# Autodesk Inventor assembly: Montagem Atualizada
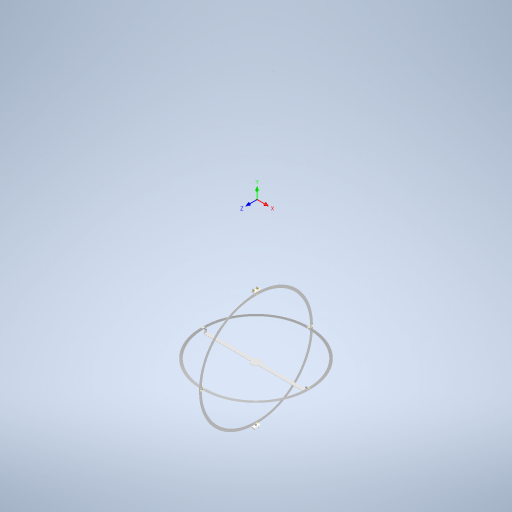
[picture p0: Inventor's stored thumbnail of the model, 512x512]
Saved by Autodesk Inventor 2024 (Build 280153000, 153)
## iProperties
Created: 2024-05-09
Part Number: Montagem Atualizada
Document SubType Name: Assembly
Designer: mathe
Author: mathe
## Documents named in this file (18)
- C:\Users\mathe\OneDrive\Área de Trabalho\Plataforma de Testes\Montagem Atualizada.iam
- C:\Users\mathe\OneDrive\Área de Trabalho\Plataforma de Testes\Suporte Central Atualizado.ipt
- C:\Users\mathe\OneDrive\Documentos\Inventor\Content Center Files\R2024\pt-BR\BS 290 SKF(19)\BS 290 SKF - SKF 108.ipt
- C:\Users\mathe\OneDrive\Área de Trabalho\Plataforma de Testes\Abraçadeira.ipt
- C:\Users\mathe\OneDrive\Área de Trabalho\Plataforma de Testes\Arco menor.ipt
- C:\Users\mathe\OneDrive\Documentos\Inventor\Content Center Files\R2024\pt-BR\BS EN 22 338  C - W\ISO 2338 - 8 h11 x 60 - CBS EN.ipt
- C:\Users\mathe\OneDrive\Documentos\Inventor\Content Center Files\R2024\pt-BR\BS 4183(5)\BS 4183 - M5 x 20(2) I.ipt
- C:\Users\mathe\OneDrive\Documentos\Inventor\Content Center Files\R2024\pt-BR\ANSI B18.2.4.2M\ANSI B18.2.4.2M - M5x0,8 - 8.ipt
- C:\Users\mathe\OneDrive\Área de Trabalho\Plataforma de Testes\Abraçadeira_CPY1.ipt
- C:\Users\mathe\OneDrive\Área de Trabalho\Plataforma de Testes\Abraçadeira_CPY1_CPY.ipt
- C:\Users\mathe\OneDrive\Área de Trabalho\Plataforma de Testes\Abraçadeira_CPY1_CPY_CPY.ipt
- C:\Users\mathe\OneDrive\Área de Trabalho\Plataforma de Testes\Arco médio.ipt
- C:\Users\mathe\OneDrive\Área de Trabalho\Plataforma de Testes\Abraçadeira_CPY1_CPY_CPY1.ipt
- C:\Users\mathe\OneDrive\Área de Trabalho\Plataforma de Testes\Abraçadeira_CPY1_CPY_CPY1_CPY.ipt
- C:\Users\mathe\OneDrive\Área de Trabalho\Plataforma de Testes\Suporte para estrutura_CPY.ipt
- C:\Users\mathe\OneDrive\Área de Trabalho\Plataforma de Testes\Pecinha do perfil.ipt
- C:\Users\mathe\OneDrive\Área de Trabalho\Plataforma de Testes\Suporte para estrutura_CPY_CPY1.ipt
- C:\Users\mathe\OneDrive\Área de Trabalho\Plataforma de Testes\Pecinha do perfil_CPY.ipt
## Components (73 placed, 17 different names)
1. Suporte Central Atualizado:1 — Coincidente:1, Coincidente:4, Coincidente:5, Coincidente:9, Coincidente:66, Coincidente:71, Ângulo:1
2. BS 290 SKF- com furo cilíndrico SKF 108:1 — Coincidente:1, Coincidente:3, Coincidente:70
3. BS 290 SKF- com furo cilíndrico SKF 108:2 — Coincidente:5, Coincidente:66, Coincidente:67
4. Abraçadeira:1 — Coincidente:7, Coincidente:8, Coincidente:10, Coincidente:11, Coincidente:13, Coincidente:14, Coincidente:15, Coincidente:17, Coincidente:18, Coincidente:19, Coincidente:20, Coincidente:21, Coincidente:65, Coincidente:70
5. BS 290 SKF- com furo cilíndrico SKF 108:3 — Coincidente:3, Coincidente:4
6. Arco menor:1 — Coincidente:7, Coincidente:8, Coincidente:17, Coincidente:47, Coincidente:48
7. BS EN 22338 C - extraído 8 h11 x 60 - C:1 — Coincidente:9, Coincidente:65
8. BS 4183 Parafuso de fenda de máquina de cabeça cilíndrica - Métrica M5 x 20:2 — Coincidente:10, Coincidente:11, Coincidente:12
9. ANSI B18.2.4.2M M5x0,8:1 — Coincidente:12, Coincidente:13
10. Arco menor:2 — Coincidente:33, Coincidente:34, Coincidente:49, Coincidente:50
11. Arco menor:3 — Coincidente:35, Coincidente:36, Coincidente:61, Coincidente:63, Ângulo:2
12. Arco menor:4 — Coincidente:14, Coincidente:15, Coincidente:18, Coincidente:62, Coincidente:64
13. BS 4183 Parafuso de fenda de máquina de cabeça cilíndrica - Métrica M5 x 20:3 — Coincidente:19, Coincidente:20, Coincidente:22
14. ANSI B18.2.4.2M M5x0,8:2 — Coincidente:21, Coincidente:22
15. BS 290 SKF- com furo cilíndrico SKF 108:4 — Coincidente:23, Coincidente:24, Coincidente:68
16. Abraçadeira_CPY1:1 — Coincidente:23, Coincidente:24, Coincidente:25, Coincidente:26, Coincidente:27, Coincidente:29, Coincidente:30, Coincidente:32, Coincidente:34, Coincidente:36, Coincidente:69, Coincidente:71
17. BS 4183 Parafuso de fenda de máquina de cabeça cilíndrica - Métrica M5 x 20:4 — Coincidente:25, Coincidente:26, Coincidente:28, Coincidente:33
18. ANSI B18.2.4.2M M5x0,8:3 — Coincidente:27, Coincidente:28
19. BS 4183 Parafuso de fenda de máquina de cabeça cilíndrica - Métrica M5 x 20:5 — Coincidente:29, Coincidente:30, Coincidente:31, Coincidente:35
20. ANSI B18.2.4.2M M5x0,8:4 — Coincidente:31, Coincidente:32
21. BS 290 SKF- com furo cilíndrico SKF 108:5 — Coincidente:72, Coincidente:76, Coincidente:77, Coincidente:144
22. Abraçadeira_CPY1_CPY:1 — Coincidente:39, Coincidente:40, Coincidente:42, Coincidente:43, Coincidente:44, Coincidente:45, Coincidente:48, Coincidente:50, Coincidente:76, Coincidente:77, Coincidente:146
23. BS 4183 Parafuso de fenda de máquina de cabeça cilíndrica - Métrica M5 x 20:6 — Coincidente:39, Coincidente:40, Coincidente:41, Coincidente:49
24. ANSI B18.2.4.2M M5x0,8:5 — Coincidente:41, Coincidente:42
25. BS 4183 Parafuso de fenda de máquina de cabeça cilíndrica - Métrica M5 x 20:7 — Coincidente:43, Coincidente:44, Coincidente:46, Coincidente:47
26. ANSI B18.2.4.2M M5x0,8:6 — Coincidente:45, Coincidente:46
27. BS 290 SKF- com furo cilíndrico SKF 108:6 — Coincidente:51, Coincidente:52, Coincidente:145
28. Abraçadeira_CPY1_CPY_CPY:1 — Coincidente:51, Coincidente:52, Coincidente:53, Coincidente:54, Coincidente:55, Coincidente:57, Coincidente:58, Coincidente:60, Coincidente:63, Coincidente:64
29. BS 4183 Parafuso de fenda de máquina de cabeça cilíndrica - Métrica M5 x 20:8 — Coincidente:53, Coincidente:54, Coincidente:56, Coincidente:61
30. ANSI B18.2.4.2M M5x0,8:7 — Coincidente:55, Coincidente:56
31. BS 4183 Parafuso de fenda de máquina de cabeça cilíndrica - Métrica M5 x 20:9 — Coincidente:57, Coincidente:58, Coincidente:59, Coincidente:62
32. ANSI B18.2.4.2M M5x0,8:8 — Coincidente:59, Coincidente:60
33. BS EN 22338 C - extraído 8 h11 x 60 - C:2 — Coincidente:67, Coincidente:68, Coincidente:69
34. BS EN 22338 C - extraído 8 h11 x 60 - C:3 — Coincidente:72
35. Arco médio:1 — Coincidente:90, Coincidente:91, Coincidente:141, Ângulo:5
36. Arco médio:2 — Coincidente:119, Coincidente:120, Coincidente:142, Coincidente:143, Ângulo:3, Ângulo:4, Ângulo:11
37. Arco médio:3 — Coincidente:103, Coincidente:105, Coincidente:117, Coincidente:118
38. Arco médio:5 — Coincidente:88, Coincidente:89, Coincidente:102, Coincidente:104
39. BS 290 SKF- com furo cilíndrico SKF 108:7 — Coincidente:78, Coincidente:79, Coincidente:155
40. Abraçadeira_CPY1_CPY:2 — Coincidente:78, Coincidente:79, Coincidente:80, Coincidente:81, Coincidente:83, Coincidente:84, Coincidente:85, Coincidente:86, Coincidente:89, Coincidente:90, Coincidente:156
41. BS 4183 Parafuso de fenda de máquina de cabeça cilíndrica - Métrica M5 x 20:10 — Coincidente:80, Coincidente:81, Coincidente:82, Coincidente:91
42. ANSI B18.2.4.2M M5x0,8:9 — Coincidente:82, Coincidente:83
43. BS 4183 Parafuso de fenda de máquina de cabeça cilíndrica - Métrica M5 x 20:11 — Coincidente:84, Coincidente:85, Coincidente:87, Coincidente:88
44. ANSI B18.2.4.2M M5x0,8:10 — Coincidente:86, Coincidente:87
45. BS 290 SKF- com furo cilíndrico SKF 108:8 — Coincidente:92, Coincidente:93, Coincidente:145, Coincidente:148
46. Abraçadeira_CPY1_CPY_CPY1:1 — Coincidente:92, Coincidente:93, Coincidente:94, Coincidente:95, Coincidente:96, Coincidente:98, Coincidente:99, Coincidente:101, Coincidente:104, Coincidente:105, Coincidente:147
47. BS 4183 Parafuso de fenda de máquina de cabeça cilíndrica - Métrica M5 x 20:12 — Coincidente:94, Coincidente:95, Coincidente:97, Coincidente:102
48. ANSI B18.2.4.2M M5x0,8:11 — Coincidente:96, Coincidente:97
49. BS 4183 Parafuso de fenda de máquina de cabeça cilíndrica - Métrica M5 x 20:13 — Coincidente:98, Coincidente:99, Coincidente:100, Coincidente:103
50. ANSI B18.2.4.2M M5x0,8:12 — Coincidente:100, Coincidente:101
51. BS 290 SKF- com furo cilíndrico SKF 108:9 — Coincidente:121, Coincidente:122, Coincidente:172
52. Abraçadeira_CPY1_CPY_CPY1_CPY:1 — Coincidente:108, Coincidente:109, Coincidente:111, Coincidente:112, Coincidente:113, Coincidente:114, Coincidente:118, Coincidente:120, Coincidente:121, Coincidente:122, Coincidente:195
53. BS 4183 Parafuso de fenda de máquina de cabeça cilíndrica - Métrica M5 x 20:14 — Coincidente:108, Coincidente:109, Coincidente:110, Coincidente:119
54. ANSI B18.2.4.2M M5x0,8:13 — Coincidente:110, Coincidente:111
55. BS 4183 Parafuso de fenda de máquina de cabeça cilíndrica - Métrica M5 x 20:15 — Coincidente:112, Coincidente:113, Coincidente:115, Coincidente:117
56. ANSI B18.2.4.2M M5x0,8:14 — Coincidente:114, Coincidente:115
57. BS 290 SKF- com furo cilíndrico SKF 108:10 — Coincidente:123, Coincidente:124, Coincidente:144
58. Abraçadeira_CPY1_CPY_CPY1:2 — Coincidente:123, Coincidente:124, Coincidente:125, Coincidente:126, Coincidente:127, Coincidente:129, Coincidente:130, Coincidente:132, Coincidente:143, Coincidente:146
59. BS 4183 Parafuso de fenda de máquina de cabeça cilíndrica - Métrica M5 x 20:16 — Coincidente:125, Coincidente:126, Coincidente:128, Coincidente:142
60. ANSI B18.2.4.2M M5x0,8:15 — Coincidente:127, Coincidente:128
61. BS 4183 Parafuso de fenda de máquina de cabeça cilíndrica - Métrica M5 x 20:17 — Coincidente:129, Coincidente:130, Coincidente:131, Coincidente:141
62. ANSI B18.2.4.2M M5x0,8:16 — Coincidente:131, Coincidente:132
63. BS EN 22338 C - extraído 8 h11 x 60 - C:4 — Coincidente:147, Coincidente:148
64. BS 290 SKF- com furo cilíndrico SKF 108:12 — Coincidente:174, Coincidente:175, Coincidente:176
65. BS EN 22338 C - extraído 8 h11 x 60 - C:7 — Coincidente:155, Coincidente:156, Coincidente:174, Coincidente:175, Coincidente:177
66. Suporte para estrutura_CPY:2 — Coincidente:176, Coincidente:177, Ângulo:5, Coincidente:178, Coincidente:179, Ângulo:7, Coincidente:180, Coincidente:181, Ângulo:8
67. BS EN 22338 C - extraído 8 h11 x 60 - C:8 — Coincidente:172, Coincidente:187, Coincidente:190
68. Pecinha do perfil:1 — Coincidente:178, Coincidente:179, Ângulo:7
69. Pecinha do perfil:2 — Coincidente:180, Coincidente:181, Ângulo:8
70. BS 290 SKF- com furo cilíndrico SKF 108:13 — Coincidente:189, Coincidente:190, Coincidente:194
71. Suporte para estrutura_CPY_CPY1:1 — Ângulo:9, Coincidente:183, Coincidente:184, Ângulo:10, Coincidente:185, Coincidente:186, Coincidente:187, Coincidente:189, Ângulo:11, Coincidente:194, Coincidente:195
72. Pecinha do perfil_CPY:1 — Ângulo:9, Coincidente:183, Coincidente:184
73. Pecinha do perfil_CPY:2 — Ângulo:10, Coincidente:185, Coincidente:186
## Relationships (161: Mate 151, Angle 10)
- Coincidente:1 [Mate]: Suporte Central Atualizado:1 ↔ BS 290 SKF- com furo cilíndrico SKF 108:1
- Coincidente:3 [Mate]: BS 290 SKF- com furo cilíndrico SKF 108:1 ↔ BS 290 SKF- com furo cilíndrico SKF 108:3
- Coincidente:4 [Mate]: Suporte Central Atualizado:1 ↔ BS 290 SKF- com furo cilíndrico SKF 108:3
- Coincidente:5 [Mate]: Suporte Central Atualizado:1 ↔ BS 290 SKF- com furo cilíndrico SKF 108:2
- Coincidente:7 [Mate]: Abraçadeira:1 ↔ Arco menor:1
- Coincidente:8 [Mate]: Abraçadeira:1 ↔ Arco menor:1
- Coincidente:9 [Mate]: Suporte Central Atualizado:1 ↔ BS EN 22338 C - extraído 8 h11 x 60 - C:1
- Coincidente:10 [Mate]: Abraçadeira:1 ↔ BS 4183 Parafuso de fenda de máquina de cabeça cilíndrica - Métrica M5 x 20:2
- Coincidente:11 [Mate]: Abraçadeira:1 ↔ BS 4183 Parafuso de fenda de máquina de cabeça cilíndrica - Métrica M5 x 20:2
- Coincidente:12 [Mate]: BS 4183 Parafuso de fenda de máquina de cabeça cilíndrica - Métrica M5 x 20:2 ↔ ANSI B18.2.4.2M M5x0,8:1
- Coincidente:13 [Mate]: Abraçadeira:1 ↔ ANSI B18.2.4.2M M5x0,8:1
- Coincidente:14 [Mate]: Abraçadeira:1 ↔ Arco menor:4
- Coincidente:15 [Mate]: Abraçadeira:1 ↔ Arco menor:4
- Coincidente:17 [Mate]: Abraçadeira:1 ↔ Arco menor:1
- Coincidente:18 [Mate]: Abraçadeira:1 ↔ Arco menor:4
- Coincidente:19 [Mate]: Abraçadeira:1 ↔ BS 4183 Parafuso de fenda de máquina de cabeça cilíndrica - Métrica M5 x 20:3
- Coincidente:20 [Mate]: Abraçadeira:1 ↔ BS 4183 Parafuso de fenda de máquina de cabeça cilíndrica - Métrica M5 x 20:3
- Coincidente:21 [Mate]: Abraçadeira:1 ↔ ANSI B18.2.4.2M M5x0,8:2
- Coincidente:22 [Mate]: BS 4183 Parafuso de fenda de máquina de cabeça cilíndrica - Métrica M5 x 20:3 ↔ ANSI B18.2.4.2M M5x0,8:2
- Coincidente:23 [Mate]: BS 290 SKF- com furo cilíndrico SKF 108:4 ↔ Abraçadeira_CPY1:1
- Coincidente:24 [Mate]: BS 290 SKF- com furo cilíndrico SKF 108:4 ↔ Abraçadeira_CPY1:1
- Coincidente:25 [Mate]: Abraçadeira_CPY1:1 ↔ BS 4183 Parafuso de fenda de máquina de cabeça cilíndrica - Métrica M5 x 20:4
- Coincidente:26 [Mate]: Abraçadeira_CPY1:1 ↔ BS 4183 Parafuso de fenda de máquina de cabeça cilíndrica - Métrica M5 x 20:4
- Coincidente:27 [Mate]: Abraçadeira_CPY1:1 ↔ ANSI B18.2.4.2M M5x0,8:3
- Coincidente:28 [Mate]: BS 4183 Parafuso de fenda de máquina de cabeça cilíndrica - Métrica M5 x 20:4 ↔ ANSI B18.2.4.2M M5x0,8:3
- Coincidente:29 [Mate]: Abraçadeira_CPY1:1 ↔ BS 4183 Parafuso de fenda de máquina de cabeça cilíndrica - Métrica M5 x 20:5
- Coincidente:30 [Mate]: Abraçadeira_CPY1:1 ↔ BS 4183 Parafuso de fenda de máquina de cabeça cilíndrica - Métrica M5 x 20:5
- Coincidente:31 [Mate]: BS 4183 Parafuso de fenda de máquina de cabeça cilíndrica - Métrica M5 x 20:5 ↔ ANSI B18.2.4.2M M5x0,8:4
- Coincidente:32 [Mate]: Abraçadeira_CPY1:1 ↔ ANSI B18.2.4.2M M5x0,8:4
- Coincidente:33 [Mate]: Arco menor:2 ↔ BS 4183 Parafuso de fenda de máquina de cabeça cilíndrica - Métrica M5 x 20:4
- Coincidente:34 [Mate]: Arco menor:2 ↔ Abraçadeira_CPY1:1
- Coincidente:35 [Mate]: Arco menor:3 ↔ BS 4183 Parafuso de fenda de máquina de cabeça cilíndrica - Métrica M5 x 20:5
- Coincidente:36 [Mate]: Arco menor:3 ↔ Abraçadeira_CPY1:1
- Coincidente:39 [Mate]: Abraçadeira_CPY1_CPY:1 ↔ BS 4183 Parafuso de fenda de máquina de cabeça cilíndrica - Métrica M5 x 20:6
- Coincidente:40 [Mate]: Abraçadeira_CPY1_CPY:1 ↔ BS 4183 Parafuso de fenda de máquina de cabeça cilíndrica - Métrica M5 x 20:6
- Coincidente:41 [Mate]: BS 4183 Parafuso de fenda de máquina de cabeça cilíndrica - Métrica M5 x 20:6 ↔ ANSI B18.2.4.2M M5x0,8:5
- Coincidente:42 [Mate]: Abraçadeira_CPY1_CPY:1 ↔ ANSI B18.2.4.2M M5x0,8:5
- Coincidente:43 [Mate]: Abraçadeira_CPY1_CPY:1 ↔ BS 4183 Parafuso de fenda de máquina de cabeça cilíndrica - Métrica M5 x 20:7
- Coincidente:44 [Mate]: Abraçadeira_CPY1_CPY:1 ↔ BS 4183 Parafuso de fenda de máquina de cabeça cilíndrica - Métrica M5 x 20:7
- Coincidente:45 [Mate]: Abraçadeira_CPY1_CPY:1 ↔ ANSI B18.2.4.2M M5x0,8:6
- Coincidente:46 [Mate]: BS 4183 Parafuso de fenda de máquina de cabeça cilíndrica - Métrica M5 x 20:7 ↔ ANSI B18.2.4.2M M5x0,8:6
- Coincidente:47 [Mate]: Arco menor:1 ↔ BS 4183 Parafuso de fenda de máquina de cabeça cilíndrica - Métrica M5 x 20:7
- Coincidente:48 [Mate]: Arco menor:1 ↔ Abraçadeira_CPY1_CPY:1
- Coincidente:49 [Mate]: Arco menor:2 ↔ BS 4183 Parafuso de fenda de máquina de cabeça cilíndrica - Métrica M5 x 20:6
- Coincidente:50 [Mate]: Arco menor:2 ↔ Abraçadeira_CPY1_CPY:1
- Coincidente:51 [Mate]: BS 290 SKF- com furo cilíndrico SKF 108:6 ↔ Abraçadeira_CPY1_CPY_CPY:1
- Coincidente:52 [Mate]: BS 290 SKF- com furo cilíndrico SKF 108:6 ↔ Abraçadeira_CPY1_CPY_CPY:1
- Coincidente:53 [Mate]: Abraçadeira_CPY1_CPY_CPY:1 ↔ BS 4183 Parafuso de fenda de máquina de cabeça cilíndrica - Métrica M5 x 20:8
- Coincidente:54 [Mate]: Abraçadeira_CPY1_CPY_CPY:1 ↔ BS 4183 Parafuso de fenda de máquina de cabeça cilíndrica - Métrica M5 x 20:8
- Coincidente:55 [Mate]: Abraçadeira_CPY1_CPY_CPY:1 ↔ ANSI B18.2.4.2M M5x0,8:7
- Coincidente:56 [Mate]: BS 4183 Parafuso de fenda de máquina de cabeça cilíndrica - Métrica M5 x 20:8 ↔ ANSI B18.2.4.2M M5x0,8:7
- Coincidente:57 [Mate]: Abraçadeira_CPY1_CPY_CPY:1 ↔ BS 4183 Parafuso de fenda de máquina de cabeça cilíndrica - Métrica M5 x 20:9
- Coincidente:58 [Mate]: Abraçadeira_CPY1_CPY_CPY:1 ↔ BS 4183 Parafuso de fenda de máquina de cabeça cilíndrica - Métrica M5 x 20:9
- Coincidente:59 [Mate]: BS 4183 Parafuso de fenda de máquina de cabeça cilíndrica - Métrica M5 x 20:9 ↔ ANSI B18.2.4.2M M5x0,8:8
- Coincidente:60 [Mate]: Abraçadeira_CPY1_CPY_CPY:1 ↔ ANSI B18.2.4.2M M5x0,8:8
- Coincidente:61 [Mate]: Arco menor:3 ↔ BS 4183 Parafuso de fenda de máquina de cabeça cilíndrica - Métrica M5 x 20:8
- Coincidente:62 [Mate]: Arco menor:4 ↔ BS 4183 Parafuso de fenda de máquina de cabeça cilíndrica - Métrica M5 x 20:9
- Coincidente:63 [Mate]: Arco menor:3 ↔ Abraçadeira_CPY1_CPY_CPY:1
- Coincidente:64 [Mate]: Arco menor:4 ↔ Abraçadeira_CPY1_CPY_CPY:1
- Coincidente:65 [Mate]: Abraçadeira:1 ↔ BS EN 22338 C - extraído 8 h11 x 60 - C:1
- Coincidente:66 [Mate]: Suporte Central Atualizado:1 ↔ BS 290 SKF- com furo cilíndrico SKF 108:2
- Coincidente:67 [Mate]: BS 290 SKF- com furo cilíndrico SKF 108:2 ↔ BS EN 22338 C - extraído 8 h11 x 60 - C:2
- Coincidente:68 [Mate]: BS 290 SKF- com furo cilíndrico SKF 108:4 ↔ BS EN 22338 C - extraído 8 h11 x 60 - C:2
- Coincidente:69 [Mate]: Abraçadeira_CPY1:1 ↔ BS EN 22338 C - extraído 8 h11 x 60 - C:2
- Coincidente:70 [Mate]: BS 290 SKF- com furo cilíndrico SKF 108:1 ↔ Abraçadeira:1
- Coincidente:71 [Mate] (30 mm): Suporte Central Atualizado:1 ↔ Abraçadeira_CPY1:1
- Coincidente:72 [Mate]: BS 290 SKF- com furo cilíndrico SKF 108:5 ↔ BS EN 22338 C - extraído 8 h11 x 60 - C:3
- Coincidente:74 [Mate]
- Coincidente:75 [Mate]
- Ângulo:1 [Angle] (0 deg): Suporte Central Atualizado:1
- Ângulo:2 [Angle] (180 deg): Arco menor:3
- Coincidente:76 [Mate]: BS 290 SKF- com furo cilíndrico SKF 108:5 ↔ Abraçadeira_CPY1_CPY:1
- Coincidente:77 [Mate]: BS 290 SKF- com furo cilíndrico SKF 108:5 ↔ Abraçadeira_CPY1_CPY:1
- Coincidente:78 [Mate]: BS 290 SKF- com furo cilíndrico SKF 108:7 ↔ Abraçadeira_CPY1_CPY:2
- Coincidente:79 [Mate]: BS 290 SKF- com furo cilíndrico SKF 108:7 ↔ Abraçadeira_CPY1_CPY:2
- Coincidente:80 [Mate]: Abraçadeira_CPY1_CPY:2 ↔ BS 4183 Parafuso de fenda de máquina de cabeça cilíndrica - Métrica M5 x 20:10
- Coincidente:81 [Mate]: Abraçadeira_CPY1_CPY:2 ↔ BS 4183 Parafuso de fenda de máquina de cabeça cilíndrica - Métrica M5 x 20:10
- Coincidente:82 [Mate]: BS 4183 Parafuso de fenda de máquina de cabeça cilíndrica - Métrica M5 x 20:10 ↔ ANSI B18.2.4.2M M5x0,8:9
- Coincidente:83 [Mate]: Abraçadeira_CPY1_CPY:2 ↔ ANSI B18.2.4.2M M5x0,8:9
- Coincidente:84 [Mate]: Abraçadeira_CPY1_CPY:2 ↔ BS 4183 Parafuso de fenda de máquina de cabeça cilíndrica - Métrica M5 x 20:11
- Coincidente:85 [Mate]: Abraçadeira_CPY1_CPY:2 ↔ BS 4183 Parafuso de fenda de máquina de cabeça cilíndrica - Métrica M5 x 20:11
- Coincidente:86 [Mate]: Abraçadeira_CPY1_CPY:2 ↔ ANSI B18.2.4.2M M5x0,8:10
- Coincidente:87 [Mate]: BS 4183 Parafuso de fenda de máquina de cabeça cilíndrica - Métrica M5 x 20:11 ↔ ANSI B18.2.4.2M M5x0,8:10
- Coincidente:88 [Mate]: Arco médio:5 ↔ BS 4183 Parafuso de fenda de máquina de cabeça cilíndrica - Métrica M5 x 20:11
- Coincidente:89 [Mate]: Arco médio:5 ↔ Abraçadeira_CPY1_CPY:2
- Coincidente:90 [Mate]: Arco médio:1 ↔ Abraçadeira_CPY1_CPY:2
- Coincidente:91 [Mate]: Arco médio:1 ↔ BS 4183 Parafuso de fenda de máquina de cabeça cilíndrica - Métrica M5 x 20:10
- Coincidente:92 [Mate]: BS 290 SKF- com furo cilíndrico SKF 108:8 ↔ Abraçadeira_CPY1_CPY_CPY1:1
- Coincidente:93 [Mate]: BS 290 SKF- com furo cilíndrico SKF 108:8 ↔ Abraçadeira_CPY1_CPY_CPY1:1
- Coincidente:94 [Mate]: Abraçadeira_CPY1_CPY_CPY1:1 ↔ BS 4183 Parafuso de fenda de máquina de cabeça cilíndrica - Métrica M5 x 20:12
- Coincidente:95 [Mate]: Abraçadeira_CPY1_CPY_CPY1:1 ↔ BS 4183 Parafuso de fenda de máquina de cabeça cilíndrica - Métrica M5 x 20:12
- Coincidente:96 [Mate]: Abraçadeira_CPY1_CPY_CPY1:1 ↔ ANSI B18.2.4.2M M5x0,8:11
- Coincidente:97 [Mate]: BS 4183 Parafuso de fenda de máquina de cabeça cilíndrica - Métrica M5 x 20:12 ↔ ANSI B18.2.4.2M M5x0,8:11
- Coincidente:98 [Mate]: Abraçadeira_CPY1_CPY_CPY1:1 ↔ BS 4183 Parafuso de fenda de máquina de cabeça cilíndrica - Métrica M5 x 20:13
- Coincidente:99 [Mate]: Abraçadeira_CPY1_CPY_CPY1:1 ↔ BS 4183 Parafuso de fenda de máquina de cabeça cilíndrica - Métrica M5 x 20:13
- Coincidente:100 [Mate]: BS 4183 Parafuso de fenda de máquina de cabeça cilíndrica - Métrica M5 x 20:13 ↔ ANSI B18.2.4.2M M5x0,8:12
- Coincidente:101 [Mate]: Abraçadeira_CPY1_CPY_CPY1:1 ↔ ANSI B18.2.4.2M M5x0,8:12
- Coincidente:102 [Mate]: Arco médio:5 ↔ BS 4183 Parafuso de fenda de máquina de cabeça cilíndrica - Métrica M5 x 20:12
- Coincidente:103 [Mate]: Arco médio:3 ↔ BS 4183 Parafuso de fenda de máquina de cabeça cilíndrica - Métrica M5 x 20:13
- Coincidente:104 [Mate]: Arco médio:5 ↔ Abraçadeira_CPY1_CPY_CPY1:1
- Coincidente:105 [Mate]: Arco médio:3 ↔ Abraçadeira_CPY1_CPY_CPY1:1
- Coincidente:108 [Mate]: Abraçadeira_CPY1_CPY_CPY1_CPY:1 ↔ BS 4183 Parafuso de fenda de máquina de cabeça cilíndrica - Métrica M5 x 20:14
- Coincidente:109 [Mate]: Abraçadeira_CPY1_CPY_CPY1_CPY:1 ↔ BS 4183 Parafuso de fenda de máquina de cabeça cilíndrica - Métrica M5 x 20:14
- Coincidente:110 [Mate]: BS 4183 Parafuso de fenda de máquina de cabeça cilíndrica - Métrica M5 x 20:14 ↔ ANSI B18.2.4.2M M5x0,8:13
- Coincidente:111 [Mate]: Abraçadeira_CPY1_CPY_CPY1_CPY:1 ↔ ANSI B18.2.4.2M M5x0,8:13
- Coincidente:112 [Mate]: Abraçadeira_CPY1_CPY_CPY1_CPY:1 ↔ BS 4183 Parafuso de fenda de máquina de cabeça cilíndrica - Métrica M5 x 20:15
- Coincidente:113 [Mate]: Abraçadeira_CPY1_CPY_CPY1_CPY:1 ↔ BS 4183 Parafuso de fenda de máquina de cabeça cilíndrica - Métrica M5 x 20:15
- Coincidente:114 [Mate]: Abraçadeira_CPY1_CPY_CPY1_CPY:1 ↔ ANSI B18.2.4.2M M5x0,8:14
- Coincidente:115 [Mate]: BS 4183 Parafuso de fenda de máquina de cabeça cilíndrica - Métrica M5 x 20:15 ↔ ANSI B18.2.4.2M M5x0,8:14
- Coincidente:117 [Mate]: Arco médio:3 ↔ BS 4183 Parafuso de fenda de máquina de cabeça cilíndrica - Métrica M5 x 20:15
- Coincidente:118 [Mate]: Arco médio:3 ↔ Abraçadeira_CPY1_CPY_CPY1_CPY:1
- Coincidente:119 [Mate]: Arco médio:2 ↔ BS 4183 Parafuso de fenda de máquina de cabeça cilíndrica - Métrica M5 x 20:14
- Coincidente:120 [Mate]: Arco médio:2 ↔ Abraçadeira_CPY1_CPY_CPY1_CPY:1
- Coincidente:121 [Mate]: BS 290 SKF- com furo cilíndrico SKF 108:9 ↔ Abraçadeira_CPY1_CPY_CPY1_CPY:1
- Coincidente:122 [Mate]: BS 290 SKF- com furo cilíndrico SKF 108:9 ↔ Abraçadeira_CPY1_CPY_CPY1_CPY:1
- Coincidente:123 [Mate]: BS 290 SKF- com furo cilíndrico SKF 108:10 ↔ Abraçadeira_CPY1_CPY_CPY1:2
- Coincidente:124 [Mate]: BS 290 SKF- com furo cilíndrico SKF 108:10 ↔ Abraçadeira_CPY1_CPY_CPY1:2
- Coincidente:125 [Mate]: Abraçadeira_CPY1_CPY_CPY1:2 ↔ BS 4183 Parafuso de fenda de máquina de cabeça cilíndrica - Métrica M5 x 20:16
- Coincidente:126 [Mate]: Abraçadeira_CPY1_CPY_CPY1:2 ↔ BS 4183 Parafuso de fenda de máquina de cabeça cilíndrica - Métrica M5 x 20:16
- Coincidente:127 [Mate]: Abraçadeira_CPY1_CPY_CPY1:2 ↔ ANSI B18.2.4.2M M5x0,8:15
- Coincidente:128 [Mate]: BS 4183 Parafuso de fenda de máquina de cabeça cilíndrica - Métrica M5 x 20:16 ↔ ANSI B18.2.4.2M M5x0,8:15
- Coincidente:129 [Mate]: Abraçadeira_CPY1_CPY_CPY1:2 ↔ BS 4183 Parafuso de fenda de máquina de cabeça cilíndrica - Métrica M5 x 20:17
- Coincidente:130 [Mate]: Abraçadeira_CPY1_CPY_CPY1:2 ↔ BS 4183 Parafuso de fenda de máquina de cabeça cilíndrica - Métrica M5 x 20:17
- Coincidente:131 [Mate]: BS 4183 Parafuso de fenda de máquina de cabeça cilíndrica - Métrica M5 x 20:17 ↔ ANSI B18.2.4.2M M5x0,8:16
- Coincidente:132 [Mate]: Abraçadeira_CPY1_CPY_CPY1:2 ↔ ANSI B18.2.4.2M M5x0,8:16
- Coincidente:141 [Mate]: Arco médio:1 ↔ BS 4183 Parafuso de fenda de máquina de cabeça cilíndrica - Métrica M5 x 20:17
- Coincidente:142 [Mate]: Arco médio:2 ↔ BS 4183 Parafuso de fenda de máquina de cabeça cilíndrica - Métrica M5 x 20:16
- Coincidente:143 [Mate]: Arco médio:2 ↔ Abraçadeira_CPY1_CPY_CPY1:2
- Coincidente:144 [Mate]: BS 290 SKF- com furo cilíndrico SKF 108:5 ↔ BS 290 SKF- com furo cilíndrico SKF 108:10
- Ângulo:3 [Angle] (90 deg): Arco médio:2
- Coincidente:145 [Mate]: BS 290 SKF- com furo cilíndrico SKF 108:6 ↔ BS 290 SKF- com furo cilíndrico SKF 108:8
- Coincidente:146 [Mate] (32.977 mm): Abraçadeira_CPY1_CPY:1 ↔ Abraçadeira_CPY1_CPY_CPY1:2
- Coincidente:147 [Mate]: Abraçadeira_CPY1_CPY_CPY1:1 ↔ BS EN 22338 C - extraído 8 h11 x 60 - C:4
- Coincidente:148 [Mate]: BS 290 SKF- com furo cilíndrico SKF 108:8 ↔ BS EN 22338 C - extraído 8 h11 x 60 - C:4
- Ângulo:4 [Angle] (0 deg): Arco médio:2
- Coincidente:155 [Mate]: BS 290 SKF- com furo cilíndrico SKF 108:7 ↔ BS EN 22338 C - extraído 8 h11 x 60 - C:7
- Coincidente:156 [Mate] (14 mm): Abraçadeira_CPY1_CPY:2 ↔ BS EN 22338 C - extraído 8 h11 x 60 - C:7
- Coincidente:172 [Mate]: BS 290 SKF- com furo cilíndrico SKF 108:9 ↔ BS EN 22338 C - extraído 8 h11 x 60 - C:8
- Coincidente:174 [Mate]: BS 290 SKF- com furo cilíndrico SKF 108:12 ↔ BS EN 22338 C - extraído 8 h11 x 60 - C:7
- Coincidente:175 [Mate]: BS 290 SKF- com furo cilíndrico SKF 108:12 ↔ BS EN 22338 C - extraído 8 h11 x 60 - C:7
- Coincidente:176 [Mate]: BS 290 SKF- com furo cilíndrico SKF 108:12 ↔ Suporte para estrutura_CPY:2
- Coincidente:177 [Mate]: BS EN 22338 C - extraído 8 h11 x 60 - C:7 ↔ Suporte para estrutura_CPY:2
- Ângulo:5 [Angle] (0 deg): Arco médio:1 ↔ Suporte para estrutura_CPY:2
- Coincidente:178 [Mate]: Suporte para estrutura_CPY:2 ↔ Pecinha do perfil:1
- Coincidente:179 [Mate]: Suporte para estrutura_CPY:2 ↔ Pecinha do perfil:1
- Ângulo:7 [Angle] (0 deg): Suporte para estrutura_CPY:2 ↔ Pecinha do perfil:1
- Coincidente:180 [Mate]: Suporte para estrutura_CPY:2 ↔ Pecinha do perfil:2
- Coincidente:181 [Mate]: Suporte para estrutura_CPY:2 ↔ Pecinha do perfil:2
- Ângulo:8 [Angle] (0 deg): Suporte para estrutura_CPY:2 ↔ Pecinha do perfil:2
- Ângulo:9 [Angle] (0 deg): Suporte para estrutura_CPY_CPY1:1 ↔ Pecinha do perfil_CPY:1
- Coincidente:183 [Mate]: Suporte para estrutura_CPY_CPY1:1 ↔ Pecinha do perfil_CPY:1
- Coincidente:184 [Mate]: Suporte para estrutura_CPY_CPY1:1 ↔ Pecinha do perfil_CPY:1
- Ângulo:10 [Angle] (0 deg): Suporte para estrutura_CPY_CPY1:1 ↔ Pecinha do perfil_CPY:2
- Coincidente:185 [Mate]: Suporte para estrutura_CPY_CPY1:1 ↔ Pecinha do perfil_CPY:2
- Coincidente:186 [Mate]: Suporte para estrutura_CPY_CPY1:1 ↔ Pecinha do perfil_CPY:2
- Coincidente:187 [Mate]: BS EN 22338 C - extraído 8 h11 x 60 - C:8 ↔ Suporte para estrutura_CPY_CPY1:1
- Coincidente:189 [Mate]: BS 290 SKF- com furo cilíndrico SKF 108:13 ↔ Suporte para estrutura_CPY_CPY1:1
- Coincidente:190 [Mate]: BS EN 22338 C - extraído 8 h11 x 60 - C:8 ↔ BS 290 SKF- com furo cilíndrico SKF 108:13
- Ângulo:11 [Angle] (0 deg): Arco médio:2 ↔ Suporte para estrutura_CPY_CPY1:1
- Coincidente:194 [Mate]: BS 290 SKF- com furo cilíndrico SKF 108:13 ↔ Suporte para estrutura_CPY_CPY1:1
- Coincidente:195 [Mate] (33.7 mm): Abraçadeira_CPY1_CPY_CPY1_CPY:1 ↔ Suporte para estrutura_CPY_CPY1:1
